# Autodesk Inventor assembly: SpeedReducerWheel
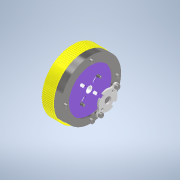
[picture p0: Inventor's stored thumbnail of the model, 180x180]
Saved by Autodesk Inventor 2021 (Build 250183000, 183)
## iProperties
Created: 2021-02-27
Part Number: SpeedReducerWheel
Document SubType Name: Assembly
Designer: Jack
Author: Jack
## Documents named in this file (37)
- C:\Users\Jack\Projekt\Wolley\MEC_SpeedReducerWheel\SpeedReducerWheel.iam
- C:\Users\Jack\Projekt\Wolley\MEC_SpeedReducerWheel\Back.ipt
- C:\Users\Jack\Projekt\Wolley\MEC_SpeedReducerWheel\RingGearA.ipt
- C:\Users\Jack\Projekt\Wolley\MEC_SpeedReducerWheel\SunGearA.ipt
- C:\Users\Jack\Projekt\Wolley\MEC_SpeedReducerWheel\PlanetGearA.ipt
- C:\Users\Jack\Projekt\Wolley\MEC_SpeedReducerWheel\Middle.ipt
- C:\Users\Jack\Projekt\Wolley\MEC_SpeedReducerWheel\PCB.ipt
- C:\Users\Jack\Projekt\Wolley\MEC_SpeedReducerWheel\Carrier.ipt
- C:\Users\Jack\Projekt\Wolley\MEC_SpeedReducerWheel\Shaft1.ipt
- C:\Users\Jack\Projekt\Wolley\MEC_SpeedReducerWheel\Shaft2.ipt
- C:\Users\Jack\Projekt\Wolley\MEC_SpeedReducerWheel\CarrierB.ipt
- C:\Users\Jack\Projekt\Wolley\MEC_SpeedReducerWheel\Front.ipt
- C:\Users\Jack\Projekt\Wolley\MEC_SpeedReducerWheel\Wheel.ipt
- C:\Users\Jack\Projekt\Wolley\MEC_SpeedReducerWheel\SunGearB.ipt
- C:\Users\Jack\Projekt\Wolley\MEC_SpeedReducerWheel\MotorPlate.ipt
- C:\Users\Jack\Projekt\Wolley\MEC_SpeedReducerWheel\Tire.ipt
- C:\Users\Jack\Projekt\Wolley\MEC_SpeedReducerWheel\Enclosure.ipt
- C:\Users\Jack\Projekt\Wolley\MEC_SpeedReducerWheel\PlanetGearB.ipt
- C:\Users\Jack\Projekt\Wolley\MEC_SpeedReducerWheel\Mount.ipt
- C:\Users\Jack\Projekt\Wolley\MEC_SpeedReducerWheel\SpeedReducerWheel\Design Accelerator\RingGearA_SpurGears.iam
- C:\Users\Jack\Projekt\Wolley\MEC_SpeedReducerWheel\SpeedReducerWheel\Design Accelerator\PlanetGearA_SpurGears2.iam
- C:\Users\Jack\Projekt\Wolley\MEC_SpeedReducerWheel\SpeedReducerWheel\Design Accelerator\SunGearB_SpurGears1.iam
- C:\Users\Jack\Projekt\Wolley\MEC_SpeedReducerWheel\SpeedReducerWheel\Design Accelerator\PlanetGearB_SpurGears1.iam
- C:\Users\Jack\Projekt\Wolley\MEC_SpeedReducerWheel\SpeedReducerWheel\Design Accelerator\RingGearB_SpurGears.iam
- C:\Users\Jack\Projekt\Wolley\MEC_SpeedReducerWheel\PlanetGearB_CPY.ipt
- C:\Users\Jack\Projekt\Wolley\MEC_SpeedReducerWheel\PlanetGearB_CPY1.ipt
- C:\Users\Jack\Documents\Inventor\Content Center Files\R2021\en-US\DIN 912\DIN 912 - M3 x 0,5 x 5 x 3,75.ipt
- C:\Users\Jack\Projekt\Wolley\MEC_SpeedReducerWheel\MiddleStandoff.ipt
- C:\Users\Jack\Projekt\Wolley\MEC_SpeedReducerWheel\SpeedReducerWheel\Design Accelerator\SunGearA_SpurGears2.iam
- C:\Users\Jack\Projekt\Wolley\MEC_SpeedReducerWheel\Shaft1_1.ipt
- C:\Users\Jack\Projekt\Wolley\MEC_SpeedReducerWheel\Magnet.ipt
- C:\Users\Jack\Projekt\Wolley\MEC_SpeedReducerWheel\Magnet_CPY.ipt
- C:\Users\Jack\Projekt\Wolley\MEC_SpeedReducerWheel\Magnet_CPY1.ipt
- C:\Users\Jack\Documents\Inventor\Content Center Files\R2021\en-US\DIN 912\DIN 912 - M3 x 0,5 x 16 x 14,75.ipt
- C:\Users\Jack\Documents\Inventor\Content Center Files\R2021\en-US\DIN 912\DIN 912 - M3 x 0,5 x 6 x 4,75.ipt
- C:\Users\Jack\Projekt\Wolley\MEC_SpeedReducerWheel\PlanetGearA_CPY2.ipt
- C:\Users\Jack\Projekt\Wolley\MEC_SpeedReducerWheel\PlanetGearA_CPY3.ipt
## Components (57 placed, 36 different names)
1. Back:1
2. RingGearA:1
3. SunGearA:1 — Flush:1, Mate:2
4. PlanetGearA:1 — Rotational:1, Flush:1
5. Middle:1 — Mate:1, Rotational:5, Rotational:6, Insert:1, Insert:2, Insert:3, Rotational:12, Rotational:13, Rotational:14, Rotational:15, Rotational:16, Rotational:17, Rotational:18
6. PCB:1 — Insert:8, Insert:9
7. Carrier:1 — Rotational:1, Rigid:2, Rigid:3, Rigid:4, Rotational:19, Rotational:20
8. Shaft1:1
9. Shaft2:1
10. CarrierB:1 — Mate:3, Mate:5, Mate:7, Rotational:9, Rotational:10, Rotational:11
11. Front:1 — Mate:4, Mate:6, Mate:8
12. Wheel:1 — Rotational:6, Rigid:1
13. SunGearB:1 — Rotational:5
14. MotorPlate:1 — Insert:10, Insert:11
15. Tire:1 — Rigid:1
16. Enclosure:1 — Insert:4, Insert:5, Insert:6, Insert:7
17. PlanetGearB:1 — Rotational:9
18. Mount:1
19. RingGearA_SpurGears:1 [sub-assembly]
20. PlanetGearA_SpurGears:1 [sub-assembly]
21. SunGearB_SpurGears:1 [sub-assembly]
22. PlanetGearB_SpurGears:1 [sub-assembly]
23. RingGearB_SpurGears:1 [sub-assembly]
24. PlanetGearB_CPY:1 — Rotational:10
25. PlanetGearB_CPY1:1 — Rotational:11
26. DIN 912 - replaced by DIN EN ISO 4762 M3 x 5:1 — Mate:3, Mate:4
27. DIN 912 - replaced by DIN EN ISO 4762 M3 x 5:2 — Mate:5, Mate:6
28. DIN 912 - replaced by DIN EN ISO 4762 M3 x 5:3 — Mate:7, Mate:8
29. DIN 912 - replaced by DIN EN ISO 4762 M3 x 5:4 — Insert:1
30. DIN 912 - replaced by DIN EN ISO 4762 M3 x 5:5 — Insert:2
31. DIN 912 - replaced by DIN EN ISO 4762 M3 x 5:6 — Insert:3
32. DIN 912 - replaced by DIN EN ISO 4762 M3 x 16:1 — Insert:4
33. DIN 912 - replaced by DIN EN ISO 4762 M3 x 16:2 — Insert:5
34. DIN 912 - replaced by DIN EN ISO 4762 M3 x 16:3 — Insert:6
35. DIN 912 - replaced by DIN EN ISO 4762 M3 x 16:4 — Insert:7
36. SunGearA_SpurGears2:1 [sub-assembly]
37. Shaft1_1:1
38. Magnet:1 — Rigid:2
39. Magnet_CPY:1 — Rigid:3
40. Magnet_CPY1:1 — Rigid:4
41. DIN 912 - replaced by DIN EN ISO 4762 M3 x 6:1 — Insert:8
42. DIN 912 - replaced by DIN EN ISO 4762 M3 x 6:2 — Insert:9
43. DIN 912 - replaced by DIN EN ISO 4762 M3 x 6:3 — Insert:10
44. DIN 912 - replaced by DIN EN ISO 4762 M3 x 6:4 — Insert:11
45. MiddleStandoff:5 — Rotational:15
46. MiddleStandoff:6 — Rotational:14
47. MiddleStandoff:7 — Rotational:13
48. MiddleStandoff:8 — Rotational:12
49. MiddleStandoff:9 — Rotational:16
50. MiddleStandoff:10 — Rotational:17
51. MiddleStandoff:11 — Rotational:18
52. PlanetGearA_CPY2:1 — Rotational:19
53. PlanetGearA_CPY3:1 — Rotational:20
54. MiddleStandoff:1
55. MiddleStandoff:2
56. MiddleStandoff:3
57. MiddleStandoff:4
## Component patterns: (4 elements, first: MiddleStandoff:1)
## Relationships (39: RevoluteJoint 15, Insert 11, Mate 8, WeldJoint 4, Flush 1)
- Rotational:1 [RevoluteJoint] (1 mm): PlanetGearA:1 ↔ Carrier:1
- Mate:1: Middle:1
- Flush:1: SunGearA:1 ↔ PlanetGearA:1
- Mate:2: SunGearA:1
- Rotational:5 [RevoluteJoint]: Middle:1 ↔ SunGearB:1
- Rotational:6 [RevoluteJoint]: Middle:1 ↔ Wheel:1
- Rigid:1 [WeldJoint]: Wheel:1 ↔ Tire:1
- Mate:3: CarrierB:1 ↔ DIN 912 - replaced by DIN EN ISO 4762 M3 x 5:1
- Mate:4: Front:1 ↔ DIN 912 - replaced by DIN EN ISO 4762 M3 x 5:1
- Mate:5: CarrierB:1 ↔ DIN 912 - replaced by DIN EN ISO 4762 M3 x 5:2
- Mate:6: Front:1 ↔ DIN 912 - replaced by DIN EN ISO 4762 M3 x 5:2
- Mate:7: CarrierB:1 ↔ DIN 912 - replaced by DIN EN ISO 4762 M3 x 5:3
- Mate:8: Front:1 ↔ DIN 912 - replaced by DIN EN ISO 4762 M3 x 5:3
- Insert:1: Middle:1 ↔ DIN 912 - replaced by DIN EN ISO 4762 M3 x 5:4
- Insert:2: Middle:1 ↔ DIN 912 - replaced by DIN EN ISO 4762 M3 x 5:5
- Insert:3: Middle:1 ↔ DIN 912 - replaced by DIN EN ISO 4762 M3 x 5:6
- Insert:4: Enclosure:1 ↔ DIN 912 - replaced by DIN EN ISO 4762 M3 x 16:1
- Insert:5: Enclosure:1 ↔ DIN 912 - replaced by DIN EN ISO 4762 M3 x 16:2
- Insert:6: Enclosure:1 ↔ DIN 912 - replaced by DIN EN ISO 4762 M3 x 16:3
- Insert:7: Enclosure:1 ↔ DIN 912 - replaced by DIN EN ISO 4762 M3 x 16:4
- Rotational:9 [RevoluteJoint]: CarrierB:1 ↔ PlanetGearB:1
- Rotational:10 [RevoluteJoint]: CarrierB:1 ↔ PlanetGearB_CPY:1
- Rotational:11 [RevoluteJoint]: CarrierB:1 ↔ PlanetGearB_CPY1:1
- Rigid:2 [WeldJoint]: Carrier:1 ↔ Magnet:1
- Rigid:3 [WeldJoint]: Carrier:1 ↔ Magnet_CPY:1
- Rigid:4 [WeldJoint]: Carrier:1 ↔ Magnet_CPY1:1
- Insert:8: PCB:1 ↔ DIN 912 - replaced by DIN EN ISO 4762 M3 x 6:1
- Insert:9: PCB:1 ↔ DIN 912 - replaced by DIN EN ISO 4762 M3 x 6:2
- Insert:10: MotorPlate:1 ↔ DIN 912 - replaced by DIN EN ISO 4762 M3 x 6:3
- Insert:11: MotorPlate:1 ↔ DIN 912 - replaced by DIN EN ISO 4762 M3 x 6:4
- Rotational:12 [RevoluteJoint]: Middle:1 ↔ MiddleStandoff:8
- Rotational:13 [RevoluteJoint]: Middle:1 ↔ MiddleStandoff:7
- Rotational:14 [RevoluteJoint]: Middle:1 ↔ MiddleStandoff:6
- Rotational:15 [RevoluteJoint]: Middle:1 ↔ MiddleStandoff:5
- Rotational:16 [RevoluteJoint]: Middle:1 ↔ MiddleStandoff:9
- Rotational:17 [RevoluteJoint]: Middle:1 ↔ MiddleStandoff:10
- Rotational:18 [RevoluteJoint]: Middle:1 ↔ MiddleStandoff:11
- Rotational:19 [RevoluteJoint]: Carrier:1 ↔ PlanetGearA_CPY2:1
- Rotational:20 [RevoluteJoint]: Carrier:1 ↔ PlanetGearA_CPY3:1
